# Autodesk Inventor assembly: assembly
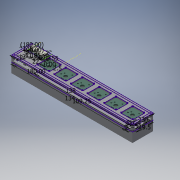
[picture p0: Inventor's stored thumbnail of the model, 180x180]
Saved by Autodesk Inventor 2017 (Build 210142000, 142)
## iProperties
Created: 2026-06-30
Part Number: assembly
Document SubType Name: Assembly
Designer: hashire umamusume
Author: hashire umamusume
## Documents named in this file (4)
- C:\Users\hashire umamusume\Documents\guilty-pad-gay\case\assembly.iam
- C:\Users\hashire umamusume\Documents\guilty-pad-gay\case\case-top.ipt
- C:\Users\hashire umamusume\Documents\guilty-pad-gay\case\pcb.iam
- C:\Users\hashire umamusume\Documents\guilty-pad-gay\case\case-bottom.ipt
## Components (3 placed, 3 different names)
1. case-top:1 — Mate:1, Flush:1, Mate:2, Flush:2, Mate:3, Flush:3, Flush:4
2. pcb:1 [sub-assembly] — Mate:1, Flush:1, Mate:2
3. case-bottom:1 — Flush:2, Mate:3, Flush:3, Flush:4
## Relationships (7: Flush 4, Mate 3)
- Mate:1: case-top:1 ↔ pcb:1
- Flush:1 (-2.54 mm): case-top:1 ↔ pcb:1
- Mate:2 (2.54 mm): case-top:1 ↔ pcb:1
- Flush:2: case-top:1 ↔ case-bottom:1
- Mate:3: case-top:1 ↔ case-bottom:1
- Flush:3: case-top:1 ↔ case-bottom:1
- Flush:4: case-top:1 ↔ case-bottom:1
